# Autodesk Inventor assembly: Elevator Sprocket with Sprockets_MIR3
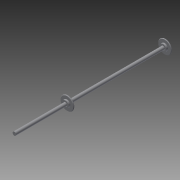
[picture p0: Inventor's stored thumbnail of the model, 180x180]
Saved by Autodesk Inventor 2015 (Build 190159000, 159)
## iProperties
Created: 2015-01-17
Part Number: Elevator Sprocket with Sprockets_MIR3
Document SubType Name: Assembly
Designer: chapale16
Author: chapale16
## Documents named in this file (3)
- H:\Elevator Sprocket with Sprockets_MIR3.iam
- H:\Elevator Axle_MIR4.ipt
- H:\Sprocket Large_MIR3.ipt
## Components (4 placed, 2 different names)
1. Elevator Axle_MIR4:1 — Flush:3, Mate:2, Mate:3
2. Sprocket Large_MIR3:1 — Flush:3, Flush:2
3. Sprocket Large_MIR3:2 — Mate:2, Flush:2, Mate:4
4. Sprocket Large_MIR3:3 — Mate:4, Mate:3
## Relationships (5: Mate 3, Flush 2)
- Flush:3: Elevator Axle_MIR4:1 ↔ Sprocket Large_MIR3:1
- Mate:2: Elevator Axle_MIR4:1 ↔ Sprocket Large_MIR3:2
- Flush:2 (361.95 mm): Sprocket Large_MIR3:1 ↔ Sprocket Large_MIR3:2
- Mate:4 (127 mm): Sprocket Large_MIR3:2 ↔ Sprocket Large_MIR3:3
- Mate:3: Elevator Axle_MIR4:1 ↔ Sprocket Large_MIR3:3
